# Autodesk Inventor assembly: 大粗轴锁轴器套
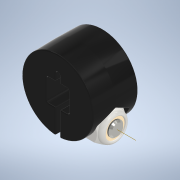
[picture p0: Inventor's stored thumbnail of the model, 180x180]
Saved by Autodesk Inventor 2020 (Build 240168000, 168)
## iProperties
Created: 2019-06-04
Part Number: 大粗轴锁轴器套
Document SubType Name: Assembly
Designer: aresp
Author: aresp
## Documents named in this file (4)
- D:\vault\ncrCadLib\轴相关\粗轴配套\大粗轴锁轴器套.iam
- D:\vault\ncrCadLib\轴相关\粗轴配套\零件\大粗轴锁轴器.ipt
- D:\vault\ncrCadLib\螺丝螺帽\Screw 8-32 x 0.625'' 四号.ipt
- D:\vault\ncrCadLib\螺丝螺帽\防滑螺帽.ipt
## Components (3 placed, 3 different names)
1. 大粗轴锁轴器:1 — 配合:1, 配合:2, 配合:4
2. Screw 8-32 x 0.625'' 四号:1 — 配合:1, 配合:2, 配合:3
3. 防滑螺帽:1 — 配合:3, 配合:4
## Relationships (4: Mate 4)
- 配合:1 [Mate]: 大粗轴锁轴器:1 ↔ Screw 8-32 x 0.625'' 四号:1
- 配合:2 [Mate]: 大粗轴锁轴器:1 ↔ Screw 8-32 x 0.625'' 四号:1
- 配合:3 [Mate]: Screw 8-32 x 0.625'' 四号:1 ↔ 防滑螺帽:1
- 配合:4 [Mate]: 大粗轴锁轴器:1 ↔ 防滑螺帽:1
